# Autodesk Inventor assembly: Y axys
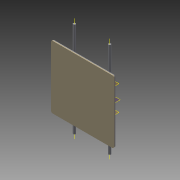
[picture p0: Inventor's stored thumbnail of the model, 180x180]
Saved by Autodesk Inventor 2014 SP1 (Build 180222100, 222)
## iProperties
Created: 2015-04-08
Part Number: Y axys
Document SubType Name: Assembly
Designer: Giorgio Nuzzo
Author: Giorgio Nuzzo
## Documents named in this file (14)
- C:\Users\Giorgio Nuzzo\Desktop\3dragmodel\Y axys.iam
- C:\Users\Giorgio Nuzzo\Desktop\3dragmodel\piastraY.ipt
- C:\Users\Giorgio Nuzzo\Desktop\3dragmodel\supporto_manicotto_X.ipt
- C:\Users\Giorgio Nuzzo\Desktop\3dragmodel\cuscinettoY.ipt
- C:\Users\Giorgio Nuzzo\Desktop\3dragmodel\supporto_manicotto_X_MIR4.ipt
- C:\Users\Giorgio Nuzzo\Desktop\3dragmodel\cuscinettoY_MIR2.ipt
- C:\Users\Giorgio Nuzzo\Desktop\3dragmodel\supporto_manicotto_X_MIR5.ipt
- C:\Users\Giorgio Nuzzo\Desktop\3dragmodel\cuscinettoY_MIR3.ipt
- C:\Users\Giorgio Nuzzo\Desktop\3dragmodel\supporto_manicotto_X_MIR4_MIR.ipt
- C:\Users\Giorgio Nuzzo\Desktop\3dragmodel\cuscinettoY_MIR2_MIR.ipt
- C:\Users\Giorgio Nuzzo\Desktop\3dragmodel\barraY.ipt
- C:\Users\Giorgio Nuzzo\Desktop\3dragmodel\barraY_MIR.ipt
- C:\Users\Giorgio Nuzzo\Desktop\3dragmodel\piastra_superiore_y.ipt
- C:\Users\Giorgio Nuzzo\Desktop\3dragmodel\piastra_superiorissima.ipt
## Components (13 placed, 13 different names)
1. piastraY:1 — Mate:1, Mate:2, Angle:1, Mate:9
2. supporto_manicotto_X:1 — Mate:2, Flush:1
3. cuscinettoY:1 — Flush:1
4. supporto_manicotto_X_MIR4:1 — Mate:3
5. cuscinettoY_MIR2:1 — Mate:3
6. supporto_manicotto_X_MIR5:1 — Mate:4
7. cuscinettoY_MIR3:1 — Mate:4
8. supporto_manicotto_X_MIR4_MIR:1 — Flush:2
9. cuscinettoY_MIR2_MIR:1 — Flush:2
10. barraY:1 — Flush:3, Mate:7
11. barraY_MIR:1 — Mate:5, Mate:6
12. piastra_superiore_y:1 — Angle:1, Mate:8, Flush:4, Mate:9, Flush:5
13. piastra_superiorissima:1 — Flush:5
## Relationships (15: Mate 9, Flush 5, Angle 1)
- Mate:1: piastraY:1
- Mate:2: piastraY:1 ↔ supporto_manicotto_X:1
- Flush:1 (-7.5 mm): supporto_manicotto_X:1 ↔ cuscinettoY:1
- Mate:3 (-7.5 mm): supporto_manicotto_X_MIR4:1 ↔ cuscinettoY_MIR2:1
- Mate:4 (-7.5 mm): supporto_manicotto_X_MIR5:1 ↔ cuscinettoY_MIR3:1
- Flush:2 (-7.5 mm): supporto_manicotto_X_MIR4_MIR:1 ↔ cuscinettoY_MIR2_MIR:1
- Flush:3: barraY:1
- Mate:5: barraY_MIR:1
- Mate:6: barraY_MIR:1
- Mate:7: barraY:1
- Angle:1 (0 deg): piastraY:1 ↔ piastra_superiore_y:1
- Mate:8: piastra_superiore_y:1
- Flush:4: piastra_superiore_y:1
- Mate:9 (10 mm): piastraY:1 ↔ piastra_superiore_y:1
- Flush:5: piastra_superiore_y:1 ↔ piastra_superiorissima:1
